# Autodesk Inventor assembly: 4_Camera
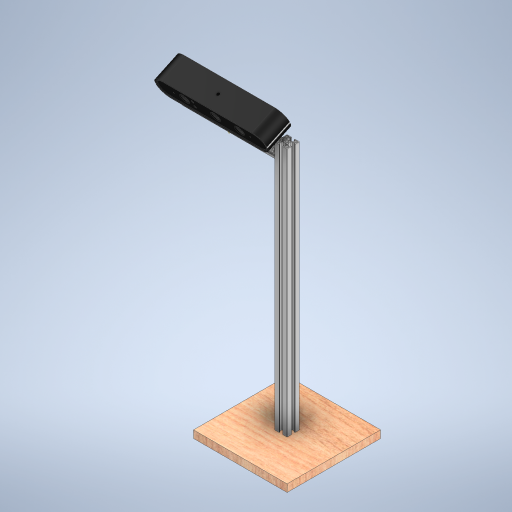
[picture p0: Inventor's stored thumbnail of the model, 512x512]
Saved by Autodesk Inventor 2024.2 (Build 282272000, 272)
## iProperties
Created: 2023-11-26
Part Number: 4_Camera
Document SubType Name: Assembly
Designer: 박동준
Author: 박동준
## Documents named in this file (5)
- C:\Users\chanh\내 드라이브\로봇\Humanoid\Roboin Humanoid Project\Inventor\rh_plus_7_axis_robot_arm_hardware\Assembly\4_Camera.iam
- C:\Users\chanh\내 드라이브\로봇\Humanoid\Roboin Humanoid Project\Inventor\rh_plus_7_axis_robot_arm_hardware\Part\Other Parts\Astra_depth_camera.ipt
- C:\Users\chanh\내 드라이브\로봇\Humanoid\Roboin Humanoid Project\Inventor\rh_plus_7_axis_robot_arm_hardware\Part\Other Parts\Aluminum_Profile_2020_400mm.ipt
- C:\Users\chanh\내 드라이브\로봇\Humanoid\Roboin Humanoid Project\Inventor\rh_plus_7_axis_robot_arm_hardware\Part\Other Parts\Aluminum_Profile_2020_150mm.ipt
- C:\Users\chanh\내 드라이브\로봇\Humanoid\Roboin Humanoid Project\Inventor\rh_plus_7_axis_robot_arm_hardware\Part\Other Parts\Camera_base_plate.ipt
## Components (4 placed, 4 different names)
1. Astra_depth_camera:1 — Mate:6, Flush:1, Mate:7
2. Aluminum_Profile_2020_400mm:1 — Mate:1, Mate:2, Angle:2, Mate:3, Angle:3, Mate:4, Mate:5, Mate:8, Angle:4, Mate:9
3. Aluminum_Profile_2020_150mm:1 — Mate:3, Angle:3, Mate:4, Mate:5, Mate:6, Flush:1, Mate:7
4. Camera_base_plate:1 — Mate:8, Angle:4, Mate:9
## Relationships (13: Mate 9, Angle 3, Flush 1)
- Mate:1: Aluminum_Profile_2020_400mm:1
- Mate:2: Aluminum_Profile_2020_400mm:1
- Angle:2 (0 deg): Aluminum_Profile_2020_400mm:1
- Mate:3: Aluminum_Profile_2020_400mm:1 ↔ Aluminum_Profile_2020_150mm:1
- Angle:3 (25 deg): Aluminum_Profile_2020_400mm:1 ↔ Aluminum_Profile_2020_150mm:1
- Mate:4: Aluminum_Profile_2020_400mm:1 ↔ Aluminum_Profile_2020_150mm:1
- Mate:5: Aluminum_Profile_2020_400mm:1 ↔ Aluminum_Profile_2020_150mm:1
- Mate:6: Astra_depth_camera:1 ↔ Aluminum_Profile_2020_150mm:1
- Flush:1 (-9 mm): Astra_depth_camera:1 ↔ Aluminum_Profile_2020_150mm:1
- Mate:7 (-75 mm): Astra_depth_camera:1 ↔ Aluminum_Profile_2020_150mm:1
- Mate:8: Aluminum_Profile_2020_400mm:1 ↔ Camera_base_plate:1
- Angle:4 (0 deg): Aluminum_Profile_2020_400mm:1 ↔ Camera_base_plate:1
- Mate:9: Aluminum_Profile_2020_400mm:1 ↔ Camera_base_plate:1
